# Autodesk Inventor assembly: RaspberriPi4B
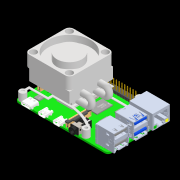
[picture p0: Inventor's stored thumbnail of the model, 180x180]
Saved by Autodesk Inventor 2020 (Build 240168000, 168)
## iProperties
Created: 2019-07-22
Part Number: RaspberriPi4B
Description: STEP AP214
Document SubType Name: Assembly
Designer: valer
Sending System: SolidWorks 2018
Preprocessor: SwSTEP 2.0
Title: Raspberry Pi 4 Model B.STEP
Revision Number: ANY
## Documents named in this file (20)
- C:\Users\valer\Desktop\drummingrobot\src\external\RaspberriPi4B.iam
- C:\Users\valer\Desktop\drummingrobot\src\external\RaspberriPi4B\PCB, RPi4ModelB.ipt
- C:\Users\valer\Desktop\drummingrobot\src\external\RaspberriPi4B\Broadcom BCM2711B0 CPU, RPi4ModelB.ipt
- C:\Users\valer\Desktop\drummingrobot\src\external\RaspberriPi4B\2.54 mm DUPONT MALE PIN HEADER, POE, 2X2, RPi4ModelB.ipt
- C:\Users\valer\Desktop\drummingrobot\src\external\RaspberriPi4B\2.54 mm DUPONT MALE PIN HEADER, IO, 2X20, RPi4ModelB.ipt
- C:\Users\valer\Desktop\drummingrobot\src\external\RaspberriPi4B\Camera Connector, RPi4ModelB.ipt
- C:\Users\valer\Desktop\drummingrobot\src\external\RaspberriPi4B\Microphone Plug, RPi4ModelB.ipt
- C:\Users\valer\Desktop\drummingrobot\src\external\RaspberriPi4B\Display Connector, RPi4ModelB.ipt
- C:\Users\valer\Desktop\drummingrobot\src\external\RaspberriPi4B\Gigabit Ethernet Port, RPi4ModelB.ipt
- C:\Users\valer\Desktop\drummingrobot\src\external\RaspberriPi4B\Female Micro HDMI Connector, RPi4ModelB.ipt
- C:\Users\valer\Desktop\drummingrobot\src\external\RaspberriPi4B\Female USB Type C Connector, RPi4ModelB.ipt
- C:\Users\valer\Desktop\drummingrobot\src\external\RaspberriPi4B\2X USB3.0 PORTS, RPi4ModelB.ipt
- C:\Users\valer\Desktop\drummingrobot\src\external\RaspberriPi4B\91D77 D9WHV 778K, 4 GB LPDDR4 SDRAM, RPi4ModelB.ipt
- C:\Users\valer\Desktop\drummingrobot\src\external\RaspberriPi4B\Cypress CYW43455 Wireless Module Cover, RPi4ModelB.ipt
- C:\Users\valer\Desktop\drummingrobot\src\external\RaspberriPi4B\SD Card Slot, RPi4ModelB.ipt
- C:\Users\valer\Desktop\drummingrobot\src\external\RaspberriPi4B\VIA VL805 PCIe USB 3.0 controller, RPi4ModelB.ipt
- C:\Users\valer\Desktop\drummingrobot\src\external\RaspberriPi4B\2X USB2.0 PORTS, RPi4ModelB.ipt
- C:\Users\valer\Desktop\drummingrobot\src\external\RaspberriPi4B\Broadcom BCM54213PE Gigabit Ethernet Transceiver, RPi4ModelB.ipt
- C:\Users\valer\Desktop\drummingrobot\src\external\RaspberriPi4B\MxL7704 Universal PMIC, RPi4ModelB.ipt
- C:\Users\valer\Desktop\drummingrobot\src\external\RaspberriPiFan.ipt
## Components (20 placed, 20 different names)
1. PCB, RPi4ModelB_1 — Mate:1, Mate:2, Mate:3
2. Broadcom BCM2711B0 CPU, RPi4ModelB_2
3. 2.54 mm DUPONT MALE PIN HEADER, POE, 2X2, RPi4ModelB_3
4. 2.54 mm DUPONT MALE PIN HEADER, IO, 2X20, RPi4ModelB_4
5. Camera Connector, RPi4ModelB_5
6. Microphone Plug, RPi4ModelB_6
7. Display Connector, RPi4ModelB_7
8. Gigabit Ethernet Port, RPi4ModelB_8
9. Female Micro HDMI Connector, RPi4ModelB_9
10. Female Micro HDMI Connector, RPi4ModelB_10
11. Female USB Type C Connector, RPi4ModelB_11
12. 2X USB3.0 PORTS, RPi4ModelB_12
13. 91D77 D9WHV 778K, 4 GB LPDDR4 SDRAM, RPi4ModelB_13
14. Cypress CYW43455 Wireless Module Cover, RPi4ModelB_14
15. SD Card Slot, RPi4ModelB_15
16. VIA VL805 PCIe USB 3.0 controller, RPi4ModelB_16
17. 2X USB2.0 PORTS, RPi4ModelB_17
18. Broadcom BCM54213PE Gigabit Ethernet Transceiver, RPi4ModelB_18
19. MxL7704 Universal PMIC, RPi4ModelB_19
20. RaspberriPiFan:1 — Mate:1, Mate:2, Mate:3
## Relationships (3: Mate 3)
- Mate:1: PCB, RPi4ModelB_1 ↔ RaspberriPiFan:1
- Mate:2: PCB, RPi4ModelB_1 ↔ RaspberriPiFan:1
- Mate:3: PCB, RPi4ModelB_1 ↔ RaspberriPiFan:1
